# Autodesk Inventor assembly: mesoSPIM_PI_M-414_Assembly_Draft_V1
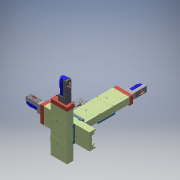
[picture p0: Inventor's stored thumbnail of the model, 180x180]
Saved by Autodesk Inventor 2019 (Build 230136000, 136)
## iProperties
Created: 2019-06-17
Part Number: mesoSPIM_PI_M-414_Assembly_Draft_V1
Document SubType Name: Assembly
Designer: voigt
Author: voigt
## Documents named in this file (6)
- D:\Microscope_Design\CAD_Files\mesoSPIM_design_V5.1\mesoSPIM\sample_stages\mesoSPIM_PI_M-414_Assembly_Draft_V1.iam
- D:\Microscope_Design\CAD_Files\mesoSPIM_design_V5.1\library\Physik_Instrumente\M-414K035_KUNDENMODELL M-414K035.ipt
- D:\Microscope_Design\CAD_Files\mesoSPIM_design_V5.1\library\Physik_Instrumente\M-414.2PD_KUNDENMODELL M-414.2PD.ipt
- D:\Microscope_Design\CAD_Files\mesoSPIM_design_V5.1\library\Physik_Instrumente\step-adapterplatten\M-413.AP2.ipt
- D:\Microscope_Design\CAD_Files\mesoSPIM_design_V5.1\library\Physik_Instrumente\step-adapterplatten\M-061.HP_00.ipt
- D:\Microscope_Design\CAD_Files\mesoSPIM_design_V5.1\library\Physik_Instrumente\M-060.DG_KUNDENMODELL.ipt
## Components (6 placed, 5 different names)
1. M-414K035_KUNDENMODELL M-414K035:1 — Mate:1, Mate:2, Mate:3, Mate:4, Mate:5
2. M-414.2PD_KUNDENMODELL M-414.2PD:1 — Mate:3, Mate:4, Mate:5, Mate:9, Mate:10, Mate:11
3. M-413.AP2:1 — Mate:6, Mate:7, Mate:8, Mate:9, Mate:10, Mate:11
4. M-414.2PD_KUNDENMODELL M-414.2PD:2 — Mate:6, Mate:7, Mate:8
5. M-061.HP_00:1
6. M-060.DG_KUNDENMODELL:1
## Relationships (11: Mate 11)
- Mate:1 (-165 mm): M-414K035_KUNDENMODELL M-414K035:1
- Mate:2: M-414K035_KUNDENMODELL M-414K035:1
- Mate:3: M-414K035_KUNDENMODELL M-414K035:1 ↔ M-414.2PD_KUNDENMODELL M-414.2PD:1
- Mate:4: M-414K035_KUNDENMODELL M-414K035:1 ↔ M-414.2PD_KUNDENMODELL M-414.2PD:1
- Mate:5: M-414K035_KUNDENMODELL M-414K035:1 ↔ M-414.2PD_KUNDENMODELL M-414.2PD:1
- Mate:6: M-413.AP2:1 ↔ M-414.2PD_KUNDENMODELL M-414.2PD:2
- Mate:7: M-413.AP2:1 ↔ M-414.2PD_KUNDENMODELL M-414.2PD:2
- Mate:8: M-413.AP2:1 ↔ M-414.2PD_KUNDENMODELL M-414.2PD:2
- Mate:9: M-414.2PD_KUNDENMODELL M-414.2PD:1 ↔ M-413.AP2:1
- Mate:10: M-414.2PD_KUNDENMODELL M-414.2PD:1 ↔ M-413.AP2:1
- Mate:11: M-414.2PD_KUNDENMODELL M-414.2PD:1 ↔ M-413.AP2:1
